# Autodesk Inventor assembly: AR-100
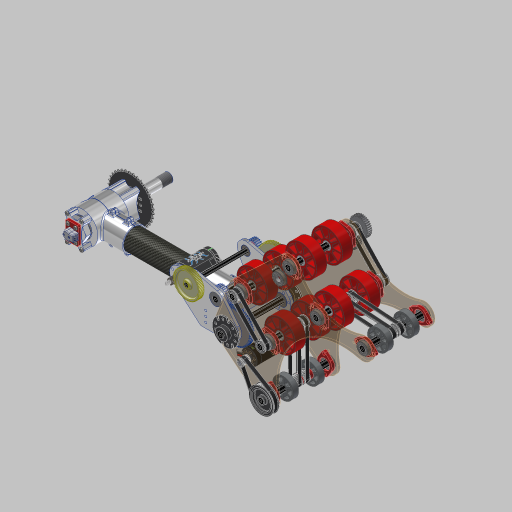
[picture p0: Inventor's stored thumbnail of the model, 512x512]
Saved by Autodesk Inventor 2023.5 (Build 275446000, 446)
## iProperties
Created: 2025-01-22
Part Number: AR-100
Document SubType Name: Assembly
Designer: slick
Mass: 4937.1 g
Surface Area: 12454.1 cm^2
Volume: 2481.98 cm^3
Density: 1.98918 g/cm^3
Author: slick
## Documents named in this file (20)
- C:\Users\slick\OneDrive\Desktop\2025-ReefScape---CAD\Arm\AR-100.iam
- C:\Users\slick\OneDrive\Desktop\2025-ReefScape---CAD\Arm\AR-001.ipt
- C:\Users\slick\OneDrive\Desktop\2025-ReefScape---CAD\COMMON PARTS\BEARINGS\0_875_ID_x_1_875_OD_X_0_500_Radial_Bearing_EE11S-2RS.ipt
- C:\Users\slick\OneDrive\Desktop\2025-ReefScape---CAD\Arm\AR-005.ipt
- C:\Users\slick\OneDrive\Desktop\2025-ReefScape---CAD\Arm\AR-006.ipt
- C:\Users\slick\OneDrive\Desktop\2025-ReefScape---CAD\COMMON PARTS\SPROCKETS\35\WCP-0983\WCP-0983.ipt
- C:\Users\slick\OneDrive\Desktop\2025-ReefScape---CAD\Arm\AR-009.ipt
- C:\Users\slick\OneDrive\Desktop\2025-ReefScape---CAD\Arm\AR-010.ipt
- C:\Users\slick\OneDrive\Desktop\2025-ReefScape---CAD\Gripper\GP3\GP3-100.iam
- C:\Users\slick\OneDrive\Desktop\2025-ReefScape---CAD\Gripper\GP4\GP4-100.iam
- C:\Users\slick\OneDrive\Desktop\2025-ReefScape---CAD\Arm\AR-013.ipt
- C:\Users\slick\OneDrive\Desktop\2025-ReefScape---CAD\Arm\AR-014.ipt
- C:\Users\slick\OneDrive\Desktop\2025-ReefScape---CAD\Elevator\EL2\EL2-A-012.ipt
- C:\Users\slick\OneDrive\Desktop\2025-ReefScape---CAD\Arm\AR-015.ipt
- C:\Users\slick\OneDrive\Desktop\2025-ReefScape---CAD\COMMON PARTS\SDS MK4i Swerve Module, 10-32, Falcons\CANcoder Assembly.iam
- C:\Users\slick\OneDrive\Desktop\2025-ReefScape---CAD\Content Center\en-US\U UNC 2605\Unbrako - 10 x 1 - 24(10).ipt
- C:\Users\slick\OneDrive\Desktop\2025-ReefScape---CAD\Content Center\en-US\U UNC 2605\Unbrako - 10 x 5_16 - 24(10).ipt
- C:\Users\slick\OneDrive\Desktop\2025-ReefScape---CAD\Content Center\en-US\U UNC 2605\Unbrako - 10 x 3_8 - 24(10).ipt
- C:\Users\slick\OneDrive\Desktop\2025-ReefScape---CAD\Gripper\GP5\GP5-100.iam
- C:\Users\slick\OneDrive\Desktop\2025-ReefScape---CAD\Gripper\GP5\GP5-300.iam
## Components (35 placed, 19 different names)
1. AR-001:1 — Mate:1, Mate:2, Mate:3, Mate:4, Mate:13, Mate:14, Insert:37, Insert:38, Insert:39, Insert:40, Insert:92
2. 0_875_ID_x_1_875_OD_X_0_500_Radial_Bearing_EE11S-2RS:1 — Mate:1, Mate:3, Mate:15, Flush:2, Mate:20
3. 0_875_ID_x_1_875_OD_X_0_500_Radial_Bearing_EE11S-2RS:2 — Mate:2, Mate:4
4. AR-005:1 — Mate:13, Mate:14, Mate:17, Mate:18, Insert:92
5. AR-006:1 — Mate:15, Flush:2, Insert:36, Mate:19, Angle:1
6. WCP-0983:1 — Insert:21, Insert:22, Insert:23, Insert:24, Insert:45, Insert:46, Insert:47, Insert:48
7. AR-009:1 — Insert:21, Insert:22, Insert:23, Insert:24, Insert:39, Insert:40
8. AR-010:1 — Mate:17, Mate:18, Insert:34, Insert:35, Insert:88, Insert:89, Insert:93, Insert:94
9. GP3-100:1 [sub-assembly]
10. GP4-100:1 [sub-assembly] — Insert:34, Insert:35, Angle:1, Insert:76, Insert:77, Insert:78, Insert:85, Insert:86, Insert:87
11. AR-013:1 — Insert:36
12. AR-014:1 — Insert:37, Insert:38, Insert:41, Insert:42, Insert:49, Insert:50, Insert:51, Insert:52
13. EL2-A-012:1 — Mate:19, Mate:20
14. AR-015:1 — Insert:41, Insert:42, Insert:43, Insert:44, Insert:53, Insert:54, Insert:55, Insert:56
15. CANcoder Assembly:1 [sub-assembly] — Insert:43, Insert:44
16. GP5-100:1 [sub-assembly] — Insert:88, Insert:89
17. GP5-300:1 [sub-assembly] — Insert:93, Insert:94
18. Unbrako UNC Hex Socket Button Cap - Inch 10 x 1:1 — Insert:45
19. Unbrako UNC Hex Socket Button Cap - Inch 10 x 1:2 — Insert:46
20. Unbrako UNC Hex Socket Button Cap - Inch 10 x 1:3 — Insert:47
21. Unbrako UNC Hex Socket Button Cap - Inch 10 x 1:4 — Insert:48
22. Unbrako UNC Hex Socket Button Cap - Inch 10 x 1:5 — Insert:49
23. Unbrako UNC Hex Socket Button Cap - Inch 10 x 1:6 — Insert:50
24. Unbrako UNC Hex Socket Button Cap - Inch 10 x 1:7 — Insert:51
25. Unbrako UNC Hex Socket Button Cap - Inch 10 x 1:8 — Insert:52
26. Unbrako UNC Hex Socket Button Cap - Inch 10 x 5/16:1 — Insert:53
27. Unbrako UNC Hex Socket Button Cap - Inch 10 x 5/16:2 — Insert:54
28. Unbrako UNC Hex Socket Button Cap - Inch 10 x 5/16:3 — Insert:55
29. Unbrako UNC Hex Socket Button Cap - Inch 10 x 5/16:4 — Insert:56
30. Unbrako UNC Hex Socket Button Cap - Inch 10 x 3/8:16 — Insert:76
31. Unbrako UNC Hex Socket Button Cap - Inch 10 x 3/8:17 — Insert:77
32. Unbrako UNC Hex Socket Button Cap - Inch 10 x 3/8:18 — Insert:78
33. Unbrako UNC Hex Socket Button Cap - Inch 10 x 3/8:25 — Insert:85
34. Unbrako UNC Hex Socket Button Cap - Inch 10 x 3/8:26 — Insert:86
35. Unbrako UNC Hex Socket Button Cap - Inch 10 x 3/8:27 — Insert:87
## Relationships (51: Insert 38, Mate 11, Flush 1, Angle 1)
- Mate:1: AR-001:1 ↔ 0_875_ID_x_1_875_OD_X_0_500_Radial_Bearing_EE11S-2RS:1
- Mate:2: AR-001:1 ↔ 0_875_ID_x_1_875_OD_X_0_500_Radial_Bearing_EE11S-2RS:2
- Mate:3: AR-001:1 ↔ 0_875_ID_x_1_875_OD_X_0_500_Radial_Bearing_EE11S-2RS:1
- Mate:4: AR-001:1 ↔ 0_875_ID_x_1_875_OD_X_0_500_Radial_Bearing_EE11S-2RS:2
- Mate:13: AR-001:1 ↔ AR-005:1
- Mate:14 (-50.8 mm): AR-001:1 ↔ AR-005:1
- Mate:15: 0_875_ID_x_1_875_OD_X_0_500_Radial_Bearing_EE11S-2RS:1 ↔ AR-006:1
- Flush:2 (-12.7 mm): 0_875_ID_x_1_875_OD_X_0_500_Radial_Bearing_EE11S-2RS:1 ↔ AR-006:1
- Insert:21: WCP-0983:1 ↔ AR-009:1
- Insert:22: WCP-0983:1 ↔ AR-009:1
- Insert:23: WCP-0983:1 ↔ AR-009:1
- Insert:24: WCP-0983:1 ↔ AR-009:1
- Mate:17: AR-005:1 ↔ AR-010:1
- Mate:18: AR-005:1 ↔ AR-010:1
- Insert:34: AR-010:1 ↔ GP4-100:1
- Insert:35: AR-010:1 ↔ GP4-100:1
- Insert:36: AR-006:1 ↔ AR-013:1
- Insert:37: AR-001:1 ↔ AR-014:1
- Insert:38: AR-001:1 ↔ AR-014:1
- Insert:39: AR-001:1 ↔ AR-009:1
- Insert:40: AR-001:1 ↔ AR-009:1
- Mate:19: AR-006:1 ↔ EL2-A-012:1
- Mate:20: 0_875_ID_x_1_875_OD_X_0_500_Radial_Bearing_EE11S-2RS:1 ↔ EL2-A-012:1
- Insert:41: AR-014:1 ↔ AR-015:1
- Insert:42: AR-014:1 ↔ AR-015:1
- Insert:43: AR-015:1 ↔ CANcoder Assembly:1
- Insert:44: AR-015:1 ↔ CANcoder Assembly:1
- Angle:1 (0 deg): AR-006:1 ↔ GP4-100:1
- Insert:45: WCP-0983:1 ↔ Unbrako UNC Hex Socket Button Cap - Inch 10 x 1:1
- Insert:46: WCP-0983:1 ↔ Unbrako UNC Hex Socket Button Cap - Inch 10 x 1:2
- Insert:47: WCP-0983:1 ↔ Unbrako UNC Hex Socket Button Cap - Inch 10 x 1:3
- Insert:48: WCP-0983:1 ↔ Unbrako UNC Hex Socket Button Cap - Inch 10 x 1:4
- Insert:49: AR-014:1 ↔ Unbrako UNC Hex Socket Button Cap - Inch 10 x 1:5
- Insert:50: AR-014:1 ↔ Unbrako UNC Hex Socket Button Cap - Inch 10 x 1:6
- Insert:51: AR-014:1 ↔ Unbrako UNC Hex Socket Button Cap - Inch 10 x 1:7
- Insert:52: AR-014:1 ↔ Unbrako UNC Hex Socket Button Cap - Inch 10 x 1:8
- Insert:53: AR-015:1 ↔ Unbrako UNC Hex Socket Button Cap - Inch 10 x 5/16:1
- Insert:54: AR-015:1 ↔ Unbrako UNC Hex Socket Button Cap - Inch 10 x 5/16:2
- Insert:55: AR-015:1 ↔ Unbrako UNC Hex Socket Button Cap - Inch 10 x 5/16:3
- Insert:56: AR-015:1 ↔ Unbrako UNC Hex Socket Button Cap - Inch 10 x 5/16:4
- Insert:76: GP4-100:1 ↔ Unbrako UNC Hex Socket Button Cap - Inch 10 x 3/8:16
- Insert:77: GP4-100:1 ↔ Unbrako UNC Hex Socket Button Cap - Inch 10 x 3/8:17
- Insert:78: GP4-100:1 ↔ Unbrako UNC Hex Socket Button Cap - Inch 10 x 3/8:18
- Insert:85: GP4-100:1 ↔ Unbrako UNC Hex Socket Button Cap - Inch 10 x 3/8:25
- Insert:86: GP4-100:1 ↔ Unbrako UNC Hex Socket Button Cap - Inch 10 x 3/8:26
- Insert:87: GP4-100:1 ↔ Unbrako UNC Hex Socket Button Cap - Inch 10 x 3/8:27
- Insert:88: AR-010:1 ↔ GP5-100:1
- Insert:89: AR-010:1 ↔ GP5-100:1
- Insert:92: AR-001:1 ↔ AR-005:1
- Insert:93: AR-010:1 ↔ GP5-300:1
- Insert:94: AR-010:1 ↔ GP5-300:1
